# Autodesk Inventor assembly: 4 in HiGrip Wheel
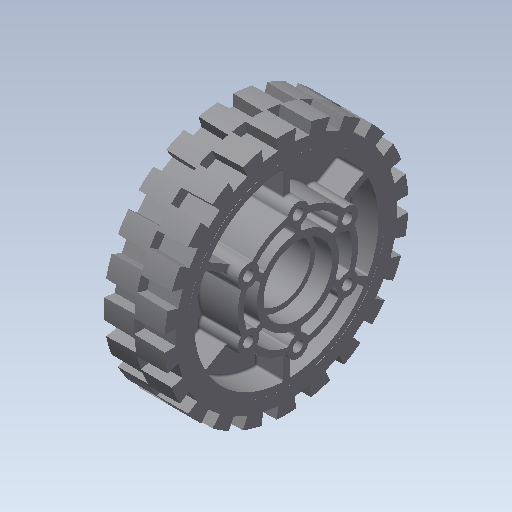
[picture p0: Inventor's stored thumbnail of the model, 512x512]
Saved by Autodesk Inventor 2020 (Build 240168000, 168)
## iProperties
Created: 2012-10-17
Part Number: 4 in HiGrip Wheel
Description: STEP AP203
Document SubType Name: Assembly
Designer: 272834E
Mass: 123.039 g
Surface Area: 761.829 cm^2
Volume: 123.039 cm^3
Density: 1 g/cm^3
Sending System: SolidWorks 2010
Preprocessor: SwSTEP 2.0
Title: 4 in HiGrip Wheel.STEP
Author: Budd
Revision Number: ANY
## Documents named in this file (3)
- C:\Users\lucky\Documents\Inventor\2020DRIVEBASE\4 in HiGrip Wheel\4 in HiGrip Wheel.iam
- C:\Users\lucky\Documents\Inventor\2020DRIVEBASE\4 in HiGrip Wheel\4 in tread.ipt
- C:\Users\lucky\Documents\Inventor\2020DRIVEBASE\4 in HiGrip Wheel\4in 2013 Hub.ipt
## Components (2 placed, 2 different names)
1. 4 in tread_1 — Mate:1, Mate:2
2. 4in 2013 Hub_2 — Mate:1, Mate:2
## Relationships (2: Mate 2)
- Mate:1: 4 in tread_1 ↔ 4in 2013 Hub_2
- Mate:2: 4 in tread_1 ↔ 4in 2013 Hub_2
